# Autodesk Inventor assembly: TestPlatform assembly
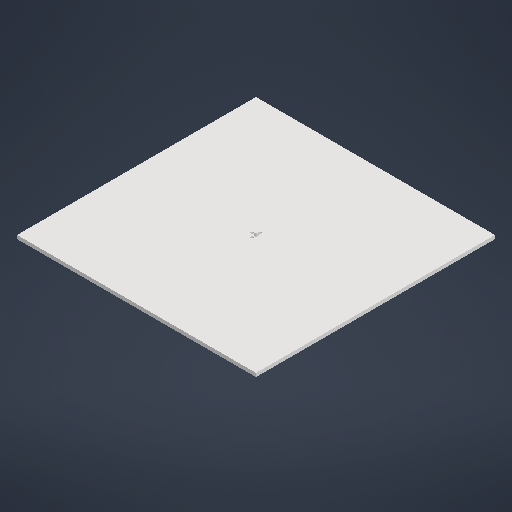
[picture p0: Inventor's stored thumbnail of the model, 512x512]
Saved by Autodesk Inventor 2026.1 (Build 301233020, 233B)
## iProperties
Created: 2025-12-03
Part Number: TestPlatform assembly
Document SubType Name: Assembly
Designer: Mikke
Author: Mikke
## Documents named in this file (5)
- C:\Users\Mikke\OneDrive - Aalborg Universitet\ESD 510 - General\Projekt\Inventor\TestPlatform\TestPlatform assembly.iam
- C:\Users\Mikke\OneDrive - Aalborg Universitet\ESD 510 - General\Projekt\Inventor\TestPlatform\Motor.ipt
- C:\Users\Mikke\OneDrive - Aalborg Universitet\ESD 510 - General\Projekt\Inventor\TestPlatform\Base stand.ipt
- C:\Users\Mikke\OneDrive - Aalborg Universitet\ESD 510 - General\Projekt\Inventor\TestPlatform\Pladeholder.ipt
- C:\Users\Mikke\OneDrive - Aalborg Universitet\ESD 510 - General\Projekt\Inventor\TestPlatform\Lasercutplade.ipt
## Components (4 placed, 4 different names)
1. Motor:1 — Flush:1, Flush:2
2. Base stand:1 — Flush:1
3. Pladeholder:1 — Flush:2, Flush:3
4. Lasercutplade:1 — Flush:3
## Relationships (3: Flush 3)
- Flush:1: Motor:1 ↔ Base stand:1
- Flush:2: Motor:1 ↔ Pladeholder:1
- Flush:3: Pladeholder:1 ↔ Lasercutplade:1
